# Autodesk Inventor assembly: 3D_Coloured_Grid
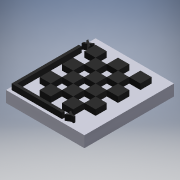
[picture p0: Inventor's stored thumbnail of the model, 180x180]
Saved by Autodesk Inventor 2019 (Build 230136000, 136)
## iProperties
Created: 2019-06-18
Part Number: 3D_Coloured_Grid
Document SubType Name: Assembly
Designer: David
Author: David
## Documents named in this file (3)
- C:\Users\David\Thesis\Breast_Cancer_Registration\3D_Models\3D_Grid_Assembly\3D_Coloured_Grid.iam
- C:\Users\David\Thesis\Breast_Cancer_Registration\3D_Models\3D_Grid_Assembly\3D_Grid_base.ipt
- C:\Users\David\Thesis\Breast_Cancer_Registration\3D_Models\3D_Grid_Assembly\3D_Grid_black_cells.ipt
## Components (2 placed, 2 different names)
1. 3D_Grid_base:1 — Rigid:1
2. 3D_Grid_black_cells:1 — Rigid:1
## Relationships (1: WeldJoint 1)
- Rigid:1 [WeldJoint]: 3D_Grid_base:1 ↔ 3D_Grid_black_cells:1
